# Autodesk Inventor assembly: 足ユニット
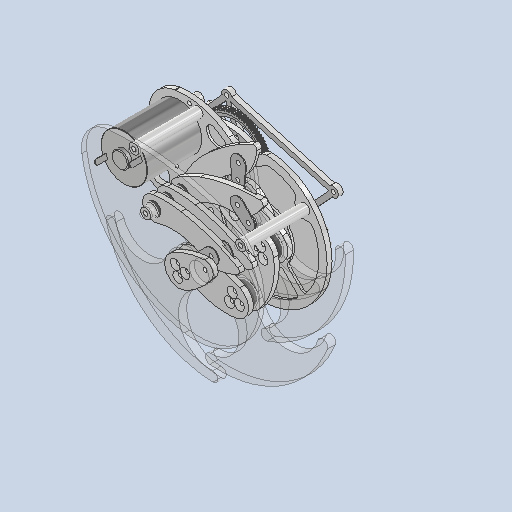
[picture p0: Inventor's stored thumbnail of the model, 512x512]
Saved by Autodesk Inventor 2022.2 (Build 262287030, 287C)
## iProperties
Created: 2022-01-10
Part Number: 足ユニット
Document SubType Name: Assembly
Designer: acps
Author: acps
## Documents named in this file (13)
- C:\Users\acps\Documents\srdc\srdc_ksh\足ユニット.iam
- C:\Users\acps\Documents\srdc\srdc_ksh\足(単独).iam
- C:\Users\acps\Documents\srdc\srdc_ksh\足外フレーム.ipt
- C:\Users\acps\Documents\srdc\srdc_ksh\足内フレーム.ipt
- C:\Users\acps\Documents\srdc\srdc_ksh\スペーサ\l40.ipt
- C:\Users\acps\Documents\srdc\srdc_ksh\ギア\脚\最終段m2z28t4.ipt
- C:\Users\acps\Documents\srdc\srdc_ksh\カム\カム4.ipt
- C:\Users\acps\Documents\srdc\srdc_ksh\オイレス\w5f15-17n.ipt
- C:\Users\acps\Documents\srdc\srdc_ksh\ギア\脚\初段_多段ギア.iam
- C:\Users\acps\Documents\srdc\srdc_ksh\モータ\M-RS-380.ipt
- C:\Users\acps\Documents\srdc\srdc_ksh\ギア\脚\ぴにょん.ipt
- C:\Users\acps\Documents\srdc\srdc_ksh\ギア抑え.ipt
- C:\Users\acps\Documents\srdc\srdc_ksh\モータマウント.ipt
## Components (14 placed, 12 different names)
1. 足外フレーム:1 — Insert:1, Mate:1, Insert:2, Insert:7
2. 足(単独):1 [sub-assembly] — Insert:1, Mate:1, Mate:2, Mate:3, Mate:5, Mate:6, Insert:6
3. 足内フレーム:1 — Mate:2, Mate:3, Mate:4, Insert:8, Mate:10, Mate:11, Mate:13, Mate:15, Mate:16, Insert:11
4. l40:1 — Insert:2
5. l40:2 — Insert:7, Insert:8
6. l40:3
7. 最終段m2z28t4:1 — Mate:7, Mate:8, Mate:9, Insert:10
8. カム4:1 — Mate:4, Mate:5, Mate:6, Insert:6, Insert:9, Mate:7, Mate:8, Mate:9, Insert:10
9. w5f15-17n:1 — Insert:9
10. 初段_多段ギア:1 [sub-assembly] — Mate:11, Mate:14
11. M-RS-380:1 — Mate:10, Mate:12
12. ぴにょん:1 — Mate:12
13. ギア抑え:1 — Mate:13, Mate:14
14. モータマウント:1 — Mate:15, Mate:16, Insert:11
## Relationships (24: Mate 16, Insert 8)
- Insert:1 (0.5 mm): 足外フレーム:1 ↔ 足(単独):1
- Mate:1: 足外フレーム:1 ↔ 足(単独):1
- Mate:2: 足(単独):1 ↔ 足内フレーム:1
- Mate:3: 足(単独):1 ↔ 足内フレーム:1
- Insert:2: 足外フレーム:1 ↔ l40:1
- Mate:4: 足内フレーム:1 ↔ カム4:1
- Mate:5: 足(単独):1 ↔ カム4:1
- Mate:6: 足(単独):1 ↔ カム4:1
- Insert:6: 足(単独):1 ↔ カム4:1
- Insert:7: 足外フレーム:1 ↔ l40:2
- Insert:8: 足内フレーム:1 ↔ l40:2
- Insert:9: カム4:1 ↔ w5f15-17n:1
- Mate:7: 最終段m2z28t4:1 ↔ カム4:1
- Mate:8: 最終段m2z28t4:1 ↔ カム4:1
- Mate:9: 最終段m2z28t4:1 ↔ カム4:1
- Insert:10: 最終段m2z28t4:1 ↔ カム4:1
- Mate:10: 足内フレーム:1 ↔ M-RS-380:1
- Mate:11: 足内フレーム:1 ↔ 初段_多段ギア:1
- Mate:12: M-RS-380:1 ↔ ぴにょん:1
- Mate:13: 足内フレーム:1 ↔ ギア抑え:1
- Mate:14: 初段_多段ギア:1 ↔ ギア抑え:1
- Mate:15: 足内フレーム:1 ↔ モータマウント:1
- Mate:16: 足内フレーム:1 ↔ モータマウント:1
- Insert:11: 足内フレーム:1 ↔ モータマウント:1
